# Autodesk Inventor assembly: TailV3
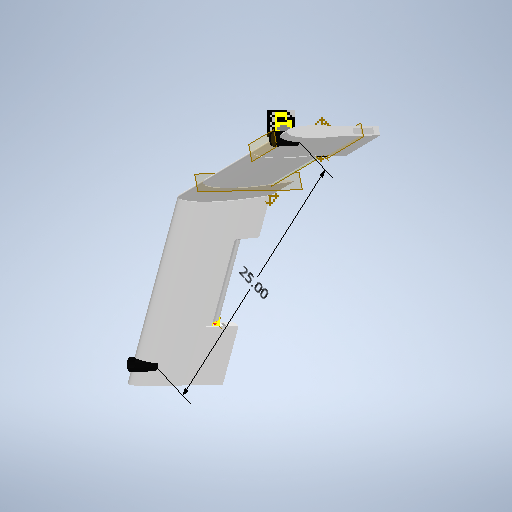
[picture p0: Inventor's stored thumbnail of the model, 512x512]
Saved by Autodesk Inventor 2025.2 (Build 292293000, 293)
## iProperties
Created: 2025-03-30
Part Number: TailV3
Document SubType Name: Assembly
Designer: georg
Author: georg
## Documents named in this file (16)
- C:\Users\georg\OneDrive\Documents\Spring 2025\Senior Design\TailV3.iam
- C:\Users\georg\OneDrive\Documents\Spring 2025\Senior Design\Tail\Part1.ipt
- C:\Users\georg\OneDrive\Documents\Spring 2025\Senior Design\MiddleTailLeft.ipt
- C:\Users\georg\OneDrive\Documents\Spring 2025\Senior Design\OuterTailLeft.ipt
- C:\Users\georg\OneDrive\Documents\Spring 2025\Senior Design\EndCap.ipt
- C:\Users\georg\OneDrive\Documents\Spring 2025\Senior Design\TailBoomReinforcement.ipt
- C:\Users\georg\Downloads\KST_DS215MG\KST_DS215MG\KST_DS215MG.ipt
- C:\Users\georg\OneDrive\Documents\Spring 2025\Senior Design\OldVersions\Elevator.ipt
- C:\Users\georg\Downloads\KST_DS215MG\25T Servo Horn Steering Arm M3\25T Servo Horn Steering Arm M3.ipt
- C:\Users\georg\OneDrive\Documents\Spring 2025\Senior Design\Tail\Part1_MIR1.ipt
- C:\Users\georg\OneDrive\Documents\Spring 2025\Senior Design\MiddleTailLeft_MIR2.ipt
- C:\Users\georg\OneDrive\Documents\Spring 2025\Senior Design\OuterTailLeft_MIR2.ipt
- C:\Users\georg\OneDrive\Documents\Spring 2025\Senior Design\TailBoomReinforcement_MIR2.ipt
- C:\Users\georg\Downloads\KST_DS215MG\KST_DS215MG\KST_DS215MG_MIR3.ipt
- C:\Users\georg\OneDrive\Documents\Spring 2025\Senior Design\OldVersions\Elevator_MIR3.ipt
- C:\Users\georg\Downloads\KST_DS215MG\25T Servo Horn Steering Arm M3\25T Servo Horn Steering Arm M3_MIR3.ipt
## Components (16 placed, 15 different names)
1. Part1:1 — Flush:2, Mate:2, Mate:3, Mate:4, Flush:3, Flush:8, Mate:30, Mate:31
2. MiddleTailLeft:1 — Flush:2, Mate:2, Mate:3, Mate:5
3. OuterTailLeft:1 — Mate:4, Flush:3, Mate:5, Mate:6, Flush:4, Mate:7, Mate:8, Mate:9, Mate:10, Mate:12, Mate:13
4. EndCap:1 — Mate:6, Flush:4, Mate:7
5. TailBoomReinforcement:1 — Mate:8, Mate:9
6. KST_DS215MG:1 — Mate:10, Mate:12, Mate:13, Cylindrical:1, Mate:14
7. Elevator:1 — Mate:15, Mate:16, Mate:17
8. 25T Servo Horn Steering Arm M3:1 — Cylindrical:1, Mate:14, Mate:15, Mate:16, Mate:17
9. Part1_MIR1:1 — Flush:8, Mate:30, Mate:31
10. MiddleTailLeft_MIR2:1 — Mate:32
11. OuterTailLeft_MIR2:1 — Mate:32, Mate:33, Mate:34, Mate:35, Mate:36, Mate:37, Mate:41, Mate:42, Flush:10
12. TailBoomReinforcement_MIR2:1 — Mate:33, Mate:34
13. KST_DS215MG_MIR3:1 — Mate:35, Mate:36, Mate:37, Mate:40, Cylindrical:2
14. Elevator_MIR3:1 — Mate:38, Mate:39, Flush:9
15. 25T Servo Horn Steering Arm M3_MIR3:1 — Mate:38, Mate:39, Flush:9, Mate:40, Cylindrical:2
16. EndCap:2 — Mate:41, Mate:42, Flush:10
## Relationships (36: Mate 28, Flush 6, CylindricalJoint 2)
- Flush:2: Part1:1 ↔ MiddleTailLeft:1
- Mate:2: Part1:1 ↔ MiddleTailLeft:1
- Mate:3: Part1:1 ↔ MiddleTailLeft:1
- Mate:4: Part1:1 ↔ OuterTailLeft:1
- Flush:3: Part1:1 ↔ OuterTailLeft:1
- Mate:5: MiddleTailLeft:1 ↔ OuterTailLeft:1
- Mate:6: OuterTailLeft:1 ↔ EndCap:1
- Flush:4: OuterTailLeft:1 ↔ EndCap:1
- Mate:7: OuterTailLeft:1 ↔ EndCap:1
- Mate:8: OuterTailLeft:1 ↔ TailBoomReinforcement:1
- Mate:9: OuterTailLeft:1 ↔ TailBoomReinforcement:1
- Mate:10: OuterTailLeft:1 ↔ KST_DS215MG:1
- Mate:12: OuterTailLeft:1 ↔ KST_DS215MG:1
- Mate:13: OuterTailLeft:1 ↔ KST_DS215MG:1
- Cylindrical:1: KST_DS215MG:1 ↔ 25T Servo Horn Steering Arm M3:1
- Mate:14: KST_DS215MG:1 ↔ 25T Servo Horn Steering Arm M3:1
- Mate:15: Elevator:1 ↔ 25T Servo Horn Steering Arm M3:1
- Mate:16: Elevator:1 ↔ 25T Servo Horn Steering Arm M3:1
- Mate:17: Elevator:1 ↔ 25T Servo Horn Steering Arm M3:1
- Flush:8: Part1:1 ↔ Part1_MIR1:1
- Mate:30: Part1:1 ↔ Part1_MIR1:1
- Mate:31: Part1:1 ↔ Part1_MIR1:1
- Mate:32: MiddleTailLeft_MIR2:1 ↔ OuterTailLeft_MIR2:1
- Mate:33: OuterTailLeft_MIR2:1 ↔ TailBoomReinforcement_MIR2:1
- Mate:34: OuterTailLeft_MIR2:1 ↔ TailBoomReinforcement_MIR2:1
- Mate:35: OuterTailLeft_MIR2:1 ↔ KST_DS215MG_MIR3:1
- Mate:36: OuterTailLeft_MIR2:1 ↔ KST_DS215MG_MIR3:1
- Mate:37: OuterTailLeft_MIR2:1 ↔ KST_DS215MG_MIR3:1
- Mate:38: Elevator_MIR3:1 ↔ 25T Servo Horn Steering Arm M3_MIR3:1
- Mate:39: Elevator_MIR3:1 ↔ 25T Servo Horn Steering Arm M3_MIR3:1
- Flush:9: Elevator_MIR3:1 ↔ 25T Servo Horn Steering Arm M3_MIR3:1
- Mate:40: KST_DS215MG_MIR3:1 ↔ 25T Servo Horn Steering Arm M3_MIR3:1
- Cylindrical:2: KST_DS215MG_MIR3:1 ↔ 25T Servo Horn Steering Arm M3_MIR3:1
- Mate:41: OuterTailLeft_MIR2:1 ↔ EndCap:2
- Mate:42: OuterTailLeft_MIR2:1 ↔ EndCap:2
- Flush:10: OuterTailLeft_MIR2:1 ↔ EndCap:2
